# Autodesk Inventor assembly: Assembly
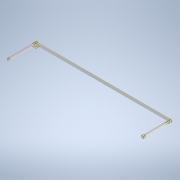
[picture p0: Inventor's stored thumbnail of the model, 180x180]
Saved by Autodesk Inventor 2022 (Build 260153000, 153)
## iProperties
Created: 2021-12-20
Part Number: Assembly
Document SubType Name: Assembly
Designer: matte
Author: matte
## Documents named in this file (6)
- C:\Users\matte\Documents\Mechanical Design Project\CAD\Assembly.iam
- C:\Users\matte\Documents\Mechanical Design Project\CAD\Parts\Elevated_track.ipt
- C:\Users\matte\Documents\Mechanical Design Project\CAD\Parts\Support_DX.ipt
- C:\Users\matte\Documents\Mechanical Design Project\CAD\Parts\Support_SX.ipt
- C:\Users\matte\Documents\Mechanical Design Project\CAD\Inventor Component Part Files\03-Brackets_Gussets_Plates\09-Machined Gussets\20-101.ipt
- C:\Users\matte\Documents\Mechanical Design Project\CAD\Inventor Component Part Files\05-Handles_Hinges\13-Pivot Joints\23-010.iam
## Components (5 placed, 5 different names)
1. Elevated_track:1 — Coincidente:1, Allineato:2, Allineato:3, Coincidente:2, Coincidente:3, Coincidente:4, Allineato:4, Coincidente:6, Coincidente:7, Allineato:5
2. Support_DX:1 — Coincidente:8, Allineato:6, Allineato:7
3. Support_SX:1 — Coincidente:1, Allineato:2, Allineato:3, Coincidente:5
4. 20-101:1 — Coincidente:4, Coincidente:5, Allineato:4
5. 23-010:1 [sub-assembly] — Coincidente:6, Coincidente:7, Allineato:5, Coincidente:8, Allineato:6, Allineato:7
## Relationships (14: Mate 8, Flush 6)
- Coincidente:1 [Mate]: Elevated_track:1 ↔ Support_SX:1
- Allineato:2 [Flush]: Elevated_track:1 ↔ Support_SX:1
- Allineato:3 [Flush]: Elevated_track:1 ↔ Support_SX:1
- Coincidente:2 [Mate]: Elevated_track:1
- Coincidente:3 [Mate]: Elevated_track:1
- Coincidente:4 [Mate]: Elevated_track:1 ↔ 20-101:1
- Coincidente:5 [Mate]: Support_SX:1 ↔ 20-101:1
- Allineato:4 [Flush]: Elevated_track:1 ↔ 20-101:1
- Coincidente:6 [Mate]: Elevated_track:1 ↔ 23-010:1
- Coincidente:7 [Mate]: Elevated_track:1 ↔ 23-010:1
- Allineato:5 [Flush]: Elevated_track:1 ↔ 23-010:1
- Coincidente:8 [Mate]: Support_DX:1 ↔ 23-010:1
- Allineato:6 [Flush]: Support_DX:1 ↔ 23-010:1
- Allineato:7 [Flush]: Support_DX:1 ↔ 23-010:1
